# Autodesk Inventor assembly: piStagesAssembly
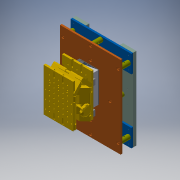
[picture p0: Inventor's stored thumbnail of the model, 180x180]
Saved by Autodesk Inventor 2016 (Build 200138000, 138)
## iProperties
Created: 2016-03-15
Part Number: piStagesAssembly
Document SubType Name: Assembly
Designer: sims01
Author: sims01
## Documents named in this file (10)
- H:\Documents\LSFM_3\setup\mechanical\design\lsfm3_mechDesign\piStagesAssembly.iam
- H:\Documents\LSFM_3\setup\mechanical\design\lsfm3_mechDesign\piStage_Z.ipt
- H:\Documents\LSFM_3\setup\mechanical\design\lsfm3_mechDesign\newportHighLoadJack.ipt
- H:\Documents\LSFM_3\setup\mechanical\design\lsfm3_mechDesign\widefieldViewingPlatformBase.ipt
- H:\Documents\LSFM_3\setup\mechanical\design\lsfm3_mechDesign\xyStageStilt.ipt
- H:\Documents\LSFM_3\setup\mechanical\design\lsfm3_mechDesign\xyStageStilt_pt2.ipt
- H:\Documents\LSFM_3\setup\mechanical\design\lsfm3_mechDesign\50mmPost.ipt
- H:\Documents\LSFM_3\setup\mechanical\design\lsfm3_mechDesign\10mmLen25mmDiamSpacer.ipt
- H:\Documents\LSFM_3\setup\mechanical\design\lsfm3_mechDesign\zStage_jackAttach.ipt
- H:\Documents\LSFM_3\setup\mechanical\design\lsfm3_mechDesign\sampleHolderAssembly.iam
## Components (20 placed, 9 different names)
1. newportHighLoadJack:1 — Rigid:38
2. piStage_Z:1 — Rigid:17, Rigid:36, Rigid:37
3. widefieldViewingPlatformBase:1 — Rigid:17, Rigid:24, Rigid:25, Rigid:26, Rigid:28, Rigid:33, Rigid:34, Rigid:35
4. xyStageStilt:1 — Rigid:21, Rigid:22
5. xyStageStilt:2 — Rigid:32, Rigid:39
6. xyStageStilt_pt2:1 — Rigid:22, Rigid:29
7. xyStageStilt_pt2:2 — Rigid:21
8. 50mmPost:1 — Rigid:30
9. 50mmPost:2 — Rigid:24
10. 50mmPost:3 — Rigid:25, Rigid:29
11. 50mmPost:4 — Rigid:26
12. 50mmPost:5 — Rigid:31
13. 50mmPost:6 — Rigid:28
14. 10mmLen25mmDiamSpacer:1 — Rigid:30, Rigid:33
15. 10mmLen25mmDiamSpacer:2 — Rigid:31, Rigid:32
16. 50mmPost:7 — Rigid:34
17. 50mmPost:8 — Rigid:35
18. zStage_jackAttach:1 — Rigid:37
19. zStage_jackAttach:2 — Rigid:36, Rigid:38
20. sampleHolderAssembly:1 [sub-assembly] — Rigid:39
## Relationships (18: WeldJoint 18)
- Rigid:17 [WeldJoint]: piStage_Z:1 ↔ widefieldViewingPlatformBase:1
- Rigid:21 [WeldJoint]: xyStageStilt:1 ↔ xyStageStilt_pt2:2
- Rigid:22 [WeldJoint]: xyStageStilt:1 ↔ xyStageStilt_pt2:1
- Rigid:24 [WeldJoint]: widefieldViewingPlatformBase:1 ↔ 50mmPost:2
- Rigid:25 [WeldJoint]: widefieldViewingPlatformBase:1 ↔ 50mmPost:3
- Rigid:26 [WeldJoint]: widefieldViewingPlatformBase:1 ↔ 50mmPost:4
- Rigid:28 [WeldJoint]: widefieldViewingPlatformBase:1 ↔ 50mmPost:6
- Rigid:29 [WeldJoint]: xyStageStilt_pt2:1 ↔ 50mmPost:3
- Rigid:30 [WeldJoint]: 50mmPost:1 ↔ 10mmLen25mmDiamSpacer:1
- Rigid:31 [WeldJoint]: 50mmPost:5 ↔ 10mmLen25mmDiamSpacer:2
- Rigid:32 [WeldJoint]: xyStageStilt:2 ↔ 10mmLen25mmDiamSpacer:2
- Rigid:33 [WeldJoint]: widefieldViewingPlatformBase:1 ↔ 10mmLen25mmDiamSpacer:1
- Rigid:34 [WeldJoint]: widefieldViewingPlatformBase:1 ↔ 50mmPost:7
- Rigid:35 [WeldJoint]: widefieldViewingPlatformBase:1 ↔ 50mmPost:8
- Rigid:36 [WeldJoint]: piStage_Z:1 ↔ zStage_jackAttach:2
- Rigid:37 [WeldJoint]: piStage_Z:1 ↔ zStage_jackAttach:1
- Rigid:38 [WeldJoint]: newportHighLoadJack:1 ↔ zStage_jackAttach:2
- Rigid:39 [WeldJoint]: xyStageStilt:2 ↔ sampleHolderAssembly:1
